# Autodesk Inventor assembly: assy
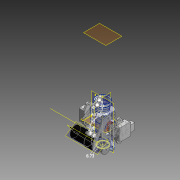
[picture p0: Inventor's stored thumbnail of the model, 180x180]
Saved by Autodesk Inventor 2015 (Build 190159000, 159)
## iProperties
Created: 2015-08-29
Part Number: assy
Document SubType Name: Assembly
Designer: francis
Mass: 406.806 g
Surface Area: 819.776 cm^2
Volume: 203.089 cm^3
Density: 2.0031 g/cm^3
Author: francis
## Documents named in this file (15)
- C:\Users\francis\Documents\GitHub\CAD\assy.iam
- C:\Users\francis\Documents\GitHub\CAD\throttle_ETC.ipt
- C:\Users\francis\Documents\GitHub\CAD\bearing.ipt
- C:\Users\francis\Documents\GitHub\CAD\crouzet_motor.ipt
- C:\Users\francis\Documents\GitHub\CAD\Bosch TPS 2\Workspaces\Workspace\Bosch TPS.ipt
- C:\Users\francis\Documents\GitHub\CAD\pulley_5mm.ipt
- C:\Users\francis\Documents\GitHub\CAD\pulley_8mm.ipt
- C:\Users\francis\Documents\GitHub\CAD\motor_plate.ipt
- C:\Users\francis\Documents\GitHub\CAD\pulley_plate.ipt
- C:\Users\francis\Documents\GitHub\CAD\spring_arm.ipt
- C:\Users\francis\Documents\Inventor\Content Center Files\R2015\en-US\ANSI B18.3.1M(6)\ANSI B18.3.1M - M4x0.7 x 10(1).ipt
- C:\Users\francis\Documents\Inventor\Content Center Files\R2015\en-US\ISO 4035(2)\ISO 4035 - M4ISO.ipt
- C:\Users\francis\Documents\Inventor\Content Center Files\R2015\en-US\ANSI B18.3.4M(1)\ANSI B18.3.4M - M4 x 0.7 x 6(2).ipt
- C:\Users\francis\Documents\Inventor\Content Center Files\R2015\en-US\ANSI B18.3.4M(1)\ANSI B18.3.4M - M3 x 0.5 x 3(2).ipt
- C:\Users\francis\Documents\Inventor\Content Center Files\R2015\en-US\ANSI B18.3.4M(1)\ANSI B18.3.4M - M3 x 0.5 x 8(2).ipt
## Components (24 placed, 14 different names)
1. throttle_ETC:1 — Mate:1, Mate:2, Mate:3, Mate:4, Mate:5, Angle:1, Angle:3, Symmetry:1, Angle:5, Flush:1, Mate:20, Mate:21, Mate:22, Flush:2, Mate:23, Flush:4, Mate:25, Mate:27, Mate:40, Mate:42, Mate:44, Mate:46, Mate:48
2. bearing:1 — Mate:2, Mate:3, Mate:6
3. bearing:2 — Mate:4, Mate:5, Mate:7, Mate:9
4. crouzet_motor:1 — Flush:1, Mate:19, Mate:21, Mate:22, Angle:6
5. Bosch TPS:1 — Angle:1, Mate:6, Mate:23
6. Bosch TPS:2 — Angle:3, Mate:7, Mate:24
7. pulley_5mm:1 — Mate:19, Flush:3
8. pulley_8mm:1 — Mate:20, Flush:3
9. motor_plate:1 — Flush:2, Mate:24
10. pulley_plate:1 — Flush:4, Mate:28, Mate:29, Insert:1, Insert:2, Mate:31, Mate:41, Mate:43, Mate:45, Mate:47, Mate:49
11. spring_arm:1 — Mate:25, Flush:27, Mate:27, Mate:36, Mate:37, Mate:38, Mate:39
12. Forged Socket Head Cap Screw - Metric M4x0.7 x 10:2 — Mate:28, Mate:29, Mate:35
13. Forged Socket Head Cap Screw - Metric M4x0.7 x 10:1 — Insert:1, Mate:30, Mate:34
14. ISO 4035 M4:4 — Insert:2
15. ISO 4035 M4:1 — Mate:30, Mate:31
16. ISO 4035 M4:3 — Mate:34
17. ISO 4035 M4:5 — Mate:35
18. Broached Hexagon Socket Button Head Cap Screw - Metric M4 x 0.7 x 6:1 — Mate:36, Mate:37
19. Broached Hexagon Socket Button Head Cap Screw - Metric M4 x 0.7 x 6:2 — Mate:38, Mate:39
20. Broached Hexagon Socket Button Head Cap Screw - Metric M3 x 0.5 x 8:1 — Mate:40, Mate:41
21. Broached Hexagon Socket Button Head Cap Screw - Metric M3 x 0.5 x 8:2 — Mate:42, Mate:43
22. Broached Hexagon Socket Button Head Cap Screw - Metric M3 x 0.5 x 3:2 — Mate:44, Mate:45
23. Broached Hexagon Socket Button Head Cap Screw - Metric M3 x 0.5 x 3:3 — Mate:46, Mate:47
24. Broached Hexagon Socket Button Head Cap Screw - Metric M3 x 0.5 x 3:4 — Mate:48, Mate:49
## Relationships (50: Mate 38, Flush 5, Angle 4, Insert 2, Symmetry 1)
- Mate:1: throttle_ETC:1
- Mate:2: throttle_ETC:1 ↔ bearing:1
- Mate:3: throttle_ETC:1 ↔ bearing:1
- Mate:4: throttle_ETC:1 ↔ bearing:2
- Mate:5: throttle_ETC:1 ↔ bearing:2
- Angle:1 (0 deg): throttle_ETC:1 ↔ Bosch TPS:1
- Angle:3 (180 deg): throttle_ETC:1 ↔ Bosch TPS:2
- Mate:6: bearing:1 ↔ Bosch TPS:1
- Mate:7: bearing:2 ↔ Bosch TPS:2
- Symmetry:1: throttle_ETC:1
- Mate:9: bearing:2
- Mate:10
- Angle:5 (90 deg): throttle_ETC:1
- Mate:13 (48.6 mm)
- Flush:1: throttle_ETC:1 ↔ crouzet_motor:1
- Mate:19: crouzet_motor:1 ↔ pulley_5mm:1
- Mate:20: throttle_ETC:1 ↔ pulley_8mm:1
- Mate:21 (48.58 mm): throttle_ETC:1 ↔ crouzet_motor:1
- Mate:22: throttle_ETC:1 ↔ crouzet_motor:1
- Angle:6 (215 deg): crouzet_motor:1
- Flush:2: throttle_ETC:1 ↔ motor_plate:1
- Flush:3: pulley_5mm:1 ↔ pulley_8mm:1
- Mate:23 (20 mm): throttle_ETC:1 ↔ Bosch TPS:1
- Mate:24 (25 mm): Bosch TPS:2 ↔ motor_plate:1
- Flush:4: throttle_ETC:1 ↔ pulley_plate:1
- Mate:25: throttle_ETC:1 ↔ spring_arm:1
- Flush:27: spring_arm:1
- Mate:27 (12 mm): throttle_ETC:1 ↔ spring_arm:1
- Mate:28: pulley_plate:1 ↔ Forged Socket Head Cap Screw - Metric M4x0.7 x 10:2
- Mate:29: pulley_plate:1 ↔ Forged Socket Head Cap Screw - Metric M4x0.7 x 10:2
- Insert:1: pulley_plate:1 ↔ Forged Socket Head Cap Screw - Metric M4x0.7 x 10:1
- Insert:2: pulley_plate:1 ↔ ISO 4035 M4:4
- Mate:30: Forged Socket Head Cap Screw - Metric M4x0.7 x 10:1 ↔ ISO 4035 M4:1
- Mate:31: pulley_plate:1 ↔ ISO 4035 M4:1
- Mate:34: Forged Socket Head Cap Screw - Metric M4x0.7 x 10:1 ↔ ISO 4035 M4:3
- Mate:35: Forged Socket Head Cap Screw - Metric M4x0.7 x 10:2 ↔ ISO 4035 M4:5
- Mate:36: spring_arm:1 ↔ Broached Hexagon Socket Button Head Cap Screw - Metric M4 x 0.7 x 6:1
- Mate:37 (5 mm): spring_arm:1 ↔ Broached Hexagon Socket Button Head Cap Screw - Metric M4 x 0.7 x 6:1
- Mate:38: spring_arm:1 ↔ Broached Hexagon Socket Button Head Cap Screw - Metric M4 x 0.7 x 6:2
- Mate:39 (5 mm): spring_arm:1 ↔ Broached Hexagon Socket Button Head Cap Screw - Metric M4 x 0.7 x 6:2
- Mate:40: throttle_ETC:1 ↔ Broached Hexagon Socket Button Head Cap Screw - Metric M3 x 0.5 x 8:1
- Mate:41: pulley_plate:1 ↔ Broached Hexagon Socket Button Head Cap Screw - Metric M3 x 0.5 x 8:1
- Mate:42: throttle_ETC:1 ↔ Broached Hexagon Socket Button Head Cap Screw - Metric M3 x 0.5 x 8:2
- Mate:43: pulley_plate:1 ↔ Broached Hexagon Socket Button Head Cap Screw - Metric M3 x 0.5 x 8:2
- Mate:44: throttle_ETC:1 ↔ Broached Hexagon Socket Button Head Cap Screw - Metric M3 x 0.5 x 3:2
- Mate:45: pulley_plate:1 ↔ Broached Hexagon Socket Button Head Cap Screw - Metric M3 x 0.5 x 3:2
- Mate:46: throttle_ETC:1 ↔ Broached Hexagon Socket Button Head Cap Screw - Metric M3 x 0.5 x 3:3
- Mate:47: pulley_plate:1 ↔ Broached Hexagon Socket Button Head Cap Screw - Metric M3 x 0.5 x 3:3
- Mate:48: throttle_ETC:1 ↔ Broached Hexagon Socket Button Head Cap Screw - Metric M3 x 0.5 x 3:4
- Mate:49: pulley_plate:1 ↔ Broached Hexagon Socket Button Head Cap Screw - Metric M3 x 0.5 x 3:4
